# Autodesk Inventor assembly: MotorClipV3
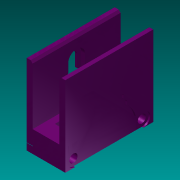
[picture p0: Inventor's stored thumbnail of the model, 180x180]
Saved by Autodesk Inventor 2013 (Build 170138000, 138)
## iProperties
Created: 2013-08-17
Part Number: MotorClipV3
Document SubType Name: Assembly
Designer: Sawaiz
Author: Sawaiz
## Documents named in this file (3)
- S:\Sawaiz\Documents\3D Modeling\Inventor\PolarGraph\MotorClipV3.iam
- S:\Sawaiz\Documents\3D Modeling\Inventor\PolarGraph\MotorClipV3Back.ipt
- S:\Sawaiz\Documents\3D Modeling\Inventor\PolarGraph\MotorClipV3Front.ipt
## Components (2 placed, 2 different names)
1. MotorClipV3Back:1 — Flush:1, Flush:2, Flush:3
2. MotorClipV3Front:1 — Flush:1, Flush:2, Flush:3
## Relationships (3: Flush 3)
- Flush:1: MotorClipV3Back:1 ↔ MotorClipV3Front:1
- Flush:2: MotorClipV3Back:1 ↔ MotorClipV3Front:1
- Flush:3: MotorClipV3Back:1 ↔ MotorClipV3Front:1
